# Autodesk Inventor assembly: 計測輪全体（回転）
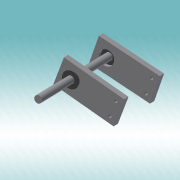
[picture p0: Inventor's stored thumbnail of the model, 180x180]
Saved by Autodesk Inventor 2015 (Build 190159000, 159)
## iProperties
Created: 2016-03-21
Part Number: 計測輪全体（回転）
Document SubType Name: Assembly
Designer: buzztaka
Author: buzztaka
## Documents named in this file (4)
- C:\Users\buzztaka\Documents\tukuba\i-cart-middle_3d-model\計測輪アセンブル\計測輪全体（回転）.iam
- C:\Users\buzztaka\Documents\tukuba\i-cart-middle_3d-model\計測輪アセンブル\回転軸取り付け板.ipt
- C:\Users\buzztaka\Documents\tukuba\i-cart-middle_3d-model\計測輪アセンブル\C-SFL6901ZZ.ipt
- C:\Users\buzztaka\Documents\tukuba\i-cart-middle_3d-model\計測輪アセンブル\回転軸.ipt
## Components (5 placed, 3 different names)
1. 回転軸取り付け板:1
2. C-SFL6901ZZ:1
3. 回転軸取り付け板:2
4. C-SFL6901ZZ:2
5. 回転軸:1
## Relationships (4: Insert 4)
- [Insert]: 回転軸取り付け板:1 ↔ C-SFL6901ZZ:1
- [Insert]: 回転軸取り付け板:2 ↔ C-SFL6901ZZ:2
- [Insert] (10 mm): C-SFL6901ZZ:2 ↔ 回転軸:1
- [Insert] (-105 mm): C-SFL6901ZZ:1 ↔ 回転軸:1
## Named parameters: d0_d2 = 10 mm, d1_d3 = -105 mm, d1_d0 = 0 mm
